# Autodesk Inventor assembly: стенка
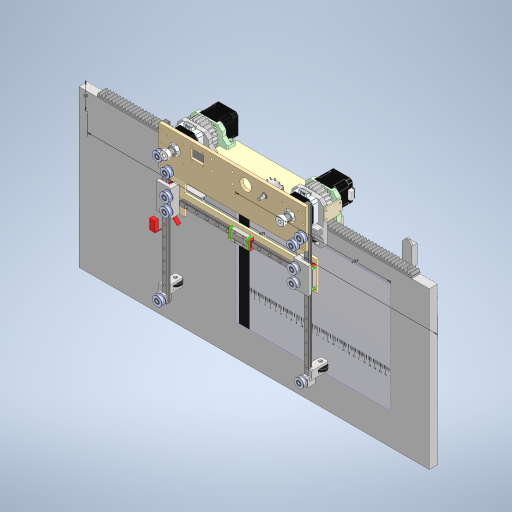
[picture p0: Inventor's stored thumbnail of the model, 512x512]
Saved by Autodesk Inventor 2023.1 (Build 271208000, 208)
## iProperties
Created: 2025-12-01
Part Number: стенка
Document SubType Name: Assembly
Designer: DELL
Author: DELL
## Documents named in this file (17)
- C:\Users\DELL\reposGitHub\VSOSH25-26\models\poligon\poligon.iam
- C:\Users\DELL\reposGitHub\VSOSH25-26\models\plotter\стенка.ipt
- C:\Users\DELL\reposGitHub\VSOSH25-26\models\import\m2_20.ipt
- C:\Users\DELL\reposGitHub\VSOSH25-26\models\poligon\poligon\Мастер проектирования\Цилиндрическое зубчатое зацепление1.iam
- C:\Users\DELL\reposGitHub\VSOSH25-26\models\poligon\poligon\Мастер проектирования\Цилиндрическое зубчатое зацепление3.iam
- C:\Users\DELL\reposGitHub\VSOSH25-26\models\poligon\poligon\Мастер проектирования\Цилиндрическое зубчатое зацепление4.iam
- C:\Users\DELL\reposGitHub\VSOSH25-26\models\poligon\poligon\Мастер проектирования\Цилиндрическое зубчатое зацепление5.iam
- C:\Users\DELL\reposGitHub\VSOSH25-26\models\poligon\poligon\Мастер проектирования\Цилиндрическое зубчатое зацепление6.iam
- C:\Users\DELL\reposGitHub\VSOSH25-26\models\poligon\poligon\Мастер проектирования\Цилиндрическое зубчатое зацепление7.iam
- C:\Users\DELL\reposGitHub\VSOSH25-26\models\actuator\actuator.iam
- C:\Users\DELL\reposGitHub\VSOSH25-26\models\plotter\plotter.iam
- C:\Users\DELL\reposGitHub\VSOSH25-26\models\actuator\лист.ipt
- C:\Users\DELL\reposGitHub\VSOSH25-26\models\plotter\plotter_new.iam
- C:\Users\DELL\reposGitHub\VSOSH25-26\models\actuator\actuator_MIR.iam
- C:\Users\DELL\reposGitHub\VSOSH25-26\models\actuator\фанера.ipt
- C:\Users\DELL\reposGitHub\VSOSH25-26\models\import\фанера_электр.ipt
- C:\Users\DELL\reposGitHub\VSOSH25-26\models\plotter\акумы.ipt
## Components (18 placed, 11 different names)
1. стенка:1 — Совмещение:1, Совмещение:2, Совмещение:4, Совмещение:6, Заподлицо:3, Совмещение:9, Совмещение:10, Совмещение:21
2. m2_20:1 — Совмещение:5, Совмещение:6
3. m2_20:2 — Совмещение:1, Совмещение:2, Совмещение:3
4. m2_20:3 — Совмещение:3, Совмещение:4, Совмещение:5, Заподлицо:1
5. Цилиндрическое зубчатое зацепление:1 [sub-assembly]
6. Цилиндрическое зубчатое зацепление:2 [sub-assembly]
7. Цилиндрическое зубчатое зацепление:3 [sub-assembly]
8. Цилиндрическое зубчатое зацепление:4 [sub-assembly]
9. Цилиндрическое зубчатое зацепление:5 [sub-assembly]
10. Цилиндрическое зубчатое зацепление:6 [sub-assembly]
11. actuator:1 [sub-assembly] — Заподлицо:1, Заподлицо:5, Совмещение:11, Совмещение:14, Совмещение:16, Совмещение:20, Совмещение:21, Заподлицо:6
12. plotter:1 [sub-assembly]
13. лист:1 — Заподлицо:3, Совмещение:9, Совмещение:10
14. plotter_new:1 [sub-assembly] — Заподлицо:5, Совмещение:11, Совмещение:14, Совмещение:15, Совмещение:19
15. actuator_MIR:1 [sub-assembly] — Совмещение:17
16. фанера:1 — Совмещение:16, Совмещение:17, Совмещение:19, Совмещение:20, Совмещение:22
17. фанера_электр:1 — Заподлицо:6
18. акумы:1 — Совмещение:22
## Relationships (21: Mate 17, Flush 4)
- Совмещение:1 [Mate] (33.5 mm): стенка:1 ↔ m2_20:2
- Совмещение:2 [Mate]: стенка:1 ↔ m2_20:2
- Совмещение:3 [Mate]: m2_20:2 ↔ m2_20:3
- Совмещение:4 [Mate]: стенка:1 ↔ m2_20:3
- Совмещение:5 [Mate]: m2_20:1 ↔ m2_20:3
- Совмещение:6 [Mate]: стенка:1 ↔ m2_20:1
- Заподлицо:1 [Flush]: m2_20:3 ↔ actuator:1
- Заподлицо:3 [Flush]: стенка:1 ↔ лист:1
- Совмещение:9 [Mate] (30 mm): стенка:1 ↔ лист:1
- Совмещение:10 [Mate] (300 mm): стенка:1 ↔ лист:1
- Заподлицо:5 [Flush]: actuator:1 ↔ plotter_new:1
- Совмещение:11 [Mate]: actuator:1 ↔ plotter_new:1
- Совмещение:14 [Mate]: actuator:1 ↔ plotter_new:1
- Совмещение:15 [Mate] (-140.4 mm): plotter_new:1
- Совмещение:16 [Mate]: actuator:1 ↔ фанера:1
- Совмещение:17 [Mate]: actuator_MIR:1 ↔ фанера:1
- Совмещение:19 [Mate]: plotter_new:1 ↔ фанера:1
- Совмещение:20 [Mate]: actuator:1 ↔ фанера:1
- Совмещение:21 [Mate] (-28.4 mm): стенка:1 ↔ actuator:1
- Заподлицо:6 [Flush]: actuator:1 ↔ фанера_электр:1
- Совмещение:22 [Mate]: фанера:1 ↔ акумы:1
